# Autodesk Inventor assembly: mirror
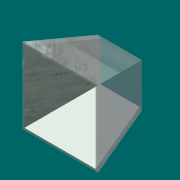
[picture p0: Inventor's stored thumbnail of the model, 180x180]
Saved by Autodesk Inventor 2016 (Build 200138000, 138)
## iProperties
Created: 2015-10-13
Part Number: mirror
Document SubType Name: Assembly
Designer: Sawaiz
Author: Sawaiz
## Documents named in this file (2)
- C:\Users\sawai\OneDrive\projects\modularRICH\mirror\mirror.iam
- C:\Users\sawai\OneDrive\projects\modularRICH\mirror\mirror.ipt
## Components (4 placed, 1 different names)
1. mirror:1 — Mate:1, Flush:1, Mate:2
2. mirror:2 — Mate:1, Flush:1, Mate:2, Mate:3, Flush:2, Mate:4
3. mirror:3 — Mate:5, Flush:3
4. mirror:4 — Mate:3, Flush:2, Mate:4, Mate:5, Flush:3
## Relationships (8: Mate 5, Flush 3)
- Mate:1: mirror:1 ↔ mirror:2
- Flush:1: mirror:1 ↔ mirror:2
- Mate:2: mirror:1 ↔ mirror:2
- Mate:3: mirror:2 ↔ mirror:4
- Flush:2: mirror:2 ↔ mirror:4
- Mate:4: mirror:2 ↔ mirror:4
- Mate:5: mirror:3 ↔ mirror:4
- Flush:3: mirror:3 ↔ mirror:4
